# Autodesk Inventor assembly: SAR330  x 5 + couplers right
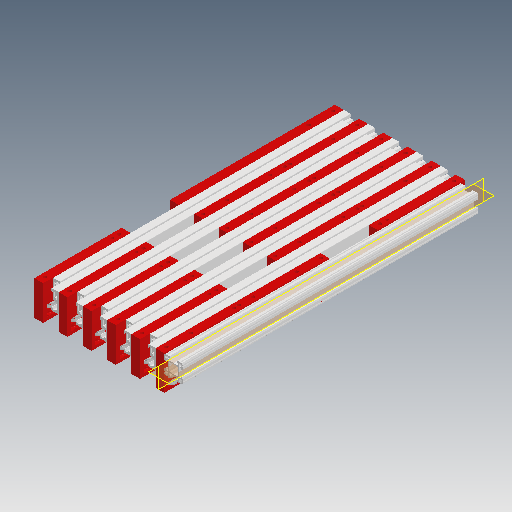
[picture p0: Inventor's stored thumbnail of the model, 512x512]
Saved by Autodesk Inventor 2020 (Build 240168000, 168)
## iProperties
Created: 2019-12-12
Part Number: SAR330  x 5 + couplers right
Document SubType Name: Assembly
Designer: ball
Author: ball
## Documents named in this file (5)
- C:\FTC\FTC8863CAD\2019 Robot\Delivery\Lift Right\SAR330  x 5 + couplers right.iam
- C:\FTC\FTC8863CAD\2019 Robot\Delivery\Lift Right\SAR330 x 4 + regular couplers right offset.iam
- C:\FTC\FTC8863CAD\2019 Robot\Delivery\Lift Right\SAR330 + fixed couplers right.iam
- C:\FTC\FTC8863CAD\2019 Robot\Delivery\Lift Right\Coupler lift short right + pulleys.iam
- C:\FTC\FTC8863CAD\2019 Robot\Delivery\Lift Right\Coupler lift long right bracket + pulley.iam
## Components (4 placed, 4 different names)
1. SAR330 x 4 + regular couplers right offset:1 [sub-assembly] — Mate:1, Mate:2, Mate:3, Mate:4, Mate:5, Mate:7, Flush:1, Mate:8, Mate:9
2. SAR330 + fixed couplers right:1 [sub-assembly] — Mate:1, Mate:2, Mate:3
3. Coupler lift short right + pulleys:1 [sub-assembly] — Mate:4, Mate:7, Flush:1
4. Coupler lift long right bracket + pulley:1 [sub-assembly] — Mate:5, Mate:8, Mate:9
## Relationships (9: Mate 8, Flush 1)
- Mate:1: SAR330 x 4 + regular couplers right offset:1 ↔ SAR330 + fixed couplers right:1
- Mate:2: SAR330 x 4 + regular couplers right offset:1 ↔ SAR330 + fixed couplers right:1
- Mate:3: SAR330 x 4 + regular couplers right offset:1 ↔ SAR330 + fixed couplers right:1
- Mate:4: SAR330 x 4 + regular couplers right offset:1 ↔ Coupler lift short right + pulleys:1
- Mate:5: SAR330 x 4 + regular couplers right offset:1 ↔ Coupler lift long right bracket + pulley:1
- Mate:7: SAR330 x 4 + regular couplers right offset:1 ↔ Coupler lift short right + pulleys:1
- Flush:1: SAR330 x 4 + regular couplers right offset:1 ↔ Coupler lift short right + pulleys:1
- Mate:8: SAR330 x 4 + regular couplers right offset:1 ↔ Coupler lift long right bracket + pulley:1
- Mate:9: SAR330 x 4 + regular couplers right offset:1 ↔ Coupler lift long right bracket + pulley:1
